# Autodesk Inventor assembly: Inner
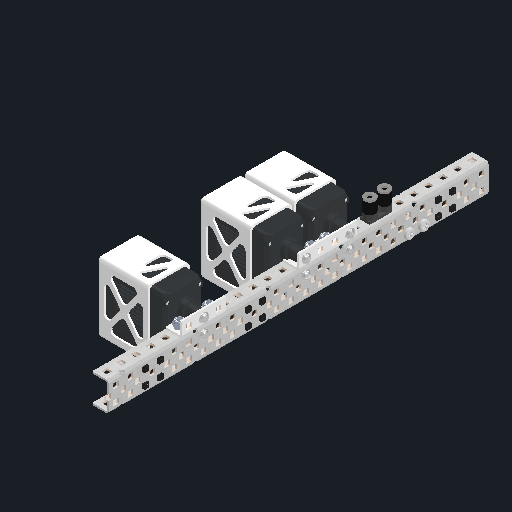
[picture p0: Inventor's stored thumbnail of the model, 512x512]
Saved by Autodesk Inventor 2025 (Build 290162000, 162)
## iProperties
Created: 2025-01-28
Part Number: Inner
Document SubType Name: Assembly
Designer: Averey Ku
Author: Averey Ku
## Documents named in this file (22)
- D:\VEX\High Stakes\CAD\V5\Chassis\Drivebay Right\Inner.iam
- D:\VEX\High Stakes\CAD\V5\Chassis\Drivebay Right\Alu C 1x2x1x26.ipt
- D:\VEX\High Stakes\CAD\V5\Chassis\Drivebay Right\Motor with Cover.iam
- D:\VEX\High Stakes\CAD\ROBOPROS-CAD-Inventor\Motion\Spacers\Washer Steel\SWasher .375 OD x .062500.ipt
- D:\VEX\High Stakes\CAD\ROBOPROS-CAD-Inventor\Motion\Spacers\Washer Steel.ipt
- D:\VEX\High Stakes\CAD\ROBOPROS-CAD-Inventor\Structure\Hardware\Screw Shoulder Robosource.ipt
- D:\VEX\High Stakes\CAD\ROBOPROS-CAD-Inventor\Structure\Hardware\Screw Shoulder Robosource\SScrew Shoulder Smooth .375 x .12.ipt
- D:\VEX\High Stakes\CAD\V5\Chassis\Drivebay Right\Nut Nylock.ipt
- D:\VEX\High Stakes\CAD\V5\Chassis\Drivebay Right\Bearing Flat Low Profile.ipt
- D:\VEX\High Stakes\CAD\V5\Chassis\Drivebay Right\NScrew Pan Head Threaded .500.ipt
- D:\VEX\High Stakes\CAD\ROBOPROS-CAD-Inventor\Structure\Hardware\Nut Nylon\Nut Nylon - White.ipt
- D:\VEX\High Stakes\CAD\ROBOPROS-CAD-Inventor\Structure\Hardware\Nut Nylon.ipt
- D:\VEX\High Stakes\CAD\V5\Chassis\Drivebay Right\4-Post Hex Nut Retainer.ipt
- D:\VEX\High Stakes\CAD\ROBOPROS-CAD-Inventor\Structure\Nylon Standoff Rounded\Nylon Standoff .875.ipt
- D:\VEX\High Stakes\CAD\ROBOPROS-CAD-Inventor\Modified Parts\Bearing Flat Low Profile 2-Hole.ipt
- D:\VEX\High Stakes\CAD\ROBOPROS-CAD-Inventor\Motion\Spacers\Spacer Nylon .375 OD\NSpacer .375 OD x .375.ipt
- D:\VEX\High Stakes\CAD\ROBOPROS-CAD-Inventor\Motion\Spacers\Spacer Nylon .375 OD.ipt
- D:\VEX\High Stakes\CAD\ROBOPROS-CAD-Inventor\Structure\Standoff\Standoff .875.ipt
- D:\VEX\High Stakes\CAD\ROBOPROS-CAD-Inventor\Structure\Standoff.ipt
- D:\VEX\High Stakes\CAD\ROBOPROS-CAD-Inventor\Structure\Hardware\Screw Alu - Slotted\AScrew Slotted Threaded .250.ipt
- D:\VEX\High Stakes\CAD\V5\Chassis\Drivebay Right\Alu C Half 1x3x1x4.ipt
- D:\VEX\High Stakes\CAD\ROBOPROS-CAD-Inventor\Structure\C Channel\Aluminum 1x3x1 Half\Alu C Half 1x3x1x3.ipt
## Components (40 placed, 16 different names)
1. Alu C 1x2x1x26:1 — Mate:1, Mate:2, Mate:3, Insert:31, Mate:8, Insert:34, Mate:9, Insert:37, Mate:10, Insert:39, Insert:37, Insert:38, Insert:39, Insert:46, Mate:11, Insert:47, Mate:12, Insert:49, Insert:50, Insert:55, Insert:61, Insert:62, Insert:63, Mate:14, Insert:64, Insert:66, Insert:70, Insert:71, Insert:72, Mate:15
2. Motor with Cover:1 [sub-assembly] — Mate:1, Insert:75
3. Motor with Cover:2 [sub-assembly] — Mate:2, Insert:73
4. Motor with Cover:3 [sub-assembly] — Mate:3, Insert:68
5. SScrew Shoulder Smooth .375 x .12:3 — Insert:64
6. Nut Nylock:1 — Insert:65
7. Bearing Flat Low Profile:1 — Insert:29, Insert:47, Mate:12, Insert:48
8. NScrew Pan Head Threaded .500:1 — Insert:31
9. Nut Nylon - White:1 — Insert:29
10. Nut Nylon - White:2 — Insert:48
11. NScrew Pan Head Threaded .500:2 — Insert:49
12. 4-Post Hex Nut Retainer:1 — Mate:8, Insert:34, Insert:35
13. Nut Nylock:2 — Insert:35
14. 4-Post Hex Nut Retainer:2 — Mate:9, Insert:37, Insert:36
15. Nut Nylock:3 — Insert:36
16. 4-Post Hex Nut Retainer:3 — Mate:10, Insert:39, Insert:38
17. Nut Nylock:4 — Insert:38
18. Nylon Standoff .875:1 — Insert:37
19. Nut Nylock:5
20. Nut Nylock:6
21. SScrew Shoulder Smooth .375 x .12:6 — Insert:38
22. SScrew Shoulder Smooth .375 x .12:7 — Insert:39
23. Bearing Flat Low Profile 2-Hole:1 — Insert:46
24. NSpacer .375 OD x .375:1
25. SWasher .375 OD x .062500:4
26. NSpacer .375 OD x .375:2 — Mate:11
27. SWasher .375 OD x .062500:5
28. Standoff .875:1 — Insert:50
29. AScrew Slotted Threaded .250:1 — Insert:76
30. AScrew Slotted Threaded .250:2 — Insert:74
31. AScrew Slotted Threaded .250:3 — Insert:55
32. Alu C Half 1x3x1x4:1 — Insert:72, Mate:15, Insert:73, Insert:74, Insert:75, Insert:76
33. AScrew Slotted Threaded .250:4 — Insert:61
34. AScrew Slotted Threaded .250:5 — Insert:62
35. Alu C Half 1x3x1x3:1 — Insert:63, Mate:14, Insert:65, Insert:67, Insert:68, Insert:69
36. SScrew Shoulder Smooth .375 x .12:8 — Insert:66
37. Nut Nylock:9 — Insert:67
38. AScrew Slotted Threaded .250:6 — Insert:70
39. AScrew Slotted Threaded .250:7 — Insert:69
40. Nylon Standoff .875:2 — Insert:71
## Relationships (47: Insert 37, Mate 10)
- Mate:1: Alu C 1x2x1x26:1 ↔ Motor with Cover:1
- Mate:2: Alu C 1x2x1x26:1 ↔ Motor with Cover:2
- Mate:3: Alu C 1x2x1x26:1 ↔ Motor with Cover:3
- Insert:31: Alu C 1x2x1x26:1 ↔ NScrew Pan Head Threaded .500:1
- Insert:29 (1.27 mm): Bearing Flat Low Profile:1 ↔ Nut Nylon - White:1
- Mate:8: Alu C 1x2x1x26:1 ↔ 4-Post Hex Nut Retainer:1
- Insert:34: Alu C 1x2x1x26:1 ↔ 4-Post Hex Nut Retainer:1
- Insert:35: 4-Post Hex Nut Retainer:1 ↔ Nut Nylock:2
- Mate:9: Alu C 1x2x1x26:1 ↔ 4-Post Hex Nut Retainer:2
- Insert:37: Alu C 1x2x1x26:1 ↔ 4-Post Hex Nut Retainer:2
- Insert:36: 4-Post Hex Nut Retainer:2 ↔ Nut Nylock:3
- Mate:10: Alu C 1x2x1x26:1 ↔ 4-Post Hex Nut Retainer:3
- Insert:39: Alu C 1x2x1x26:1 ↔ 4-Post Hex Nut Retainer:3
- Insert:38: 4-Post Hex Nut Retainer:3 ↔ Nut Nylock:4
- Insert:37: Alu C 1x2x1x26:1 ↔ Nylon Standoff .875:1
- Insert:38: Alu C 1x2x1x26:1 ↔ SScrew Shoulder Smooth .375 x .12:6
- Insert:39: Alu C 1x2x1x26:1 ↔ SScrew Shoulder Smooth .375 x .12:7
- [Insert]: NSpacer .375 OD x .375:1 ↔ SWasher .375 OD x .062500:4
- [Insert] (1.27 mm): Bearing Flat Low Profile 2-Hole:1 ↔ NSpacer .375 OD x .375:1
- [Insert]: NSpacer .375 OD x .375:2 ↔ SWasher .375 OD x .062500:5
- [Insert] (1.27 mm): Bearing Flat Low Profile 2-Hole:1 ↔ NSpacer .375 OD x .375:2
- Insert:46: Alu C 1x2x1x26:1 ↔ Bearing Flat Low Profile 2-Hole:1
- Mate:11: Alu C 1x2x1x26:1 ↔ NSpacer .375 OD x .375:2
- Insert:47: Alu C 1x2x1x26:1 ↔ Bearing Flat Low Profile:1
- Mate:12: Alu C 1x2x1x26:1 ↔ Bearing Flat Low Profile:1
- Insert:48 (1.27 mm): Bearing Flat Low Profile:1 ↔ Nut Nylon - White:2
- Insert:49: Alu C 1x2x1x26:1 ↔ NScrew Pan Head Threaded .500:2
- Insert:50: Alu C 1x2x1x26:1 ↔ Standoff .875:1
- Insert:55: Alu C 1x2x1x26:1 ↔ AScrew Slotted Threaded .250:3
- Insert:61: Alu C 1x2x1x26:1 ↔ AScrew Slotted Threaded .250:4
- Insert:62: Alu C 1x2x1x26:1 ↔ AScrew Slotted Threaded .250:5
- Insert:63: Alu C 1x2x1x26:1 ↔ Alu C Half 1x3x1x3:1
- Mate:14: Alu C 1x2x1x26:1 ↔ Alu C Half 1x3x1x3:1
- Insert:64: Alu C 1x2x1x26:1 ↔ SScrew Shoulder Smooth .375 x .12:3
- Insert:65: Nut Nylock:1 ↔ Alu C Half 1x3x1x3:1
- Insert:66: Alu C 1x2x1x26:1 ↔ SScrew Shoulder Smooth .375 x .12:8
- Insert:67: Alu C Half 1x3x1x3:1 ↔ Nut Nylock:9
- Insert:68: Motor with Cover:3 ↔ Alu C Half 1x3x1x3:1
- Insert:69: Alu C Half 1x3x1x3:1 ↔ AScrew Slotted Threaded .250:7
- Insert:70: Alu C 1x2x1x26:1 ↔ AScrew Slotted Threaded .250:6
- Insert:71: Alu C 1x2x1x26:1 ↔ Nylon Standoff .875:2
- Insert:72: Alu C 1x2x1x26:1 ↔ Alu C Half 1x3x1x4:1
- Mate:15: Alu C 1x2x1x26:1 ↔ Alu C Half 1x3x1x4:1
- Insert:73: Motor with Cover:2 ↔ Alu C Half 1x3x1x4:1
- Insert:74: AScrew Slotted Threaded .250:2 ↔ Alu C Half 1x3x1x4:1
- Insert:75: Motor with Cover:1 ↔ Alu C Half 1x3x1x4:1
- Insert:76: AScrew Slotted Threaded .250:1 ↔ Alu C Half 1x3x1x4:1
## Named parameters: d102_d100 = 0 mm
